# Autodesk Inventor assembly: Piston Bracket Assembly
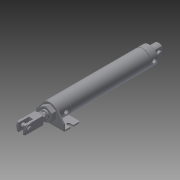
[picture p0: Inventor's stored thumbnail of the model, 180x180]
Saved by Autodesk Inventor 2013 (Build 170138000, 138)
## iProperties
Created: 2013-03-16
Part Number: Piston Bracket Assembly
Document SubType Name: Assembly
Designer: Arpan
Author: Arpan
## Documents named in this file (3)
- C:\Users\Arpan\Documents\GitHub\frc2013CAD\Midwest Climber\Piston Bracket Assembly.iam
- C:\Users\Arpan\Documents\GitHub\frc2013CAD\Midwest Climber\ninja cylinder foot bracket.ipt
- C:\Users\Arpan\Documents\GitHub\frc2013CAD\Midwest Climber\good piston.iam
## Components (2 placed, 2 different names)
1. ninja cylinder foot bracket:1 — Mate:1, Mate:2, Angle:1
2. good piston:1 [sub-assembly] — Mate:1, Mate:2, Angle:1
## Relationships (3: Mate 2, Angle 1)
- Mate:1: ninja cylinder foot bracket:1 ↔ good piston:1
- Mate:2: ninja cylinder foot bracket:1 ↔ good piston:1
- Angle:1 (0 deg): ninja cylinder foot bracket:1 ↔ good piston:1
